# Autodesk Inventor assembly: JewlArm
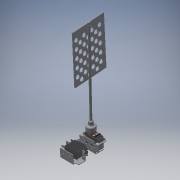
[picture p0: Inventor's stored thumbnail of the model, 180x180]
Saved by Autodesk Inventor 2017 (Build 210142000, 142)
## iProperties
Created: 2017-10-12
Part Number: JewlArm
Document SubType Name: Assembly
Designer: User
Author: User
## Documents named in this file (5)
- C:\Robotics\CAD\2017-18_CAD\Miscellaneous\JewlArm.iam
- C:\Robotics\CAD\COTSParts\Tetrix\Tetrix servo 180.ipt
- C:\Robotics\CAD\COTSParts\Tetrix\Tetrix bracket - single servo.ipt
- C:\Robotics\CAD\2017-18_CAD\FlapperSlapperPlate.ipt
- C:\Robotics\CAD\2017-18_CAD\FlapperSlapper.ipt
## Components (6 placed, 4 different names)
1. Tetrix servo 180:1 — Mate:11, Mate:12, Mate:13, Mate:21, Mate:22
2. Tetrix servo 180:2 — Mate:10, Mate:18, Mate:19, Mate:20
3. Tetrix bracket - single servo:1 — Mate:18, Mate:19, Mate:20, Flush:1, Flush:2
4. Tetrix bracket - single servo:2 — Mate:10, Mate:11, Mate:12, Mate:13, Flush:1, Flush:2
5. FlapperSlapperPlate:1 — Mate:23, Mate:24
6. FlapperSlapper:1 — Mate:21, Mate:22, Mate:23, Mate:24
## Relationships (13: Mate 11, Flush 2)
- Mate:10 (10.668 mm): Tetrix servo 180:2 ↔ Tetrix bracket - single servo:2
- Mate:11: Tetrix servo 180:1 ↔ Tetrix bracket - single servo:2
- Mate:12: Tetrix servo 180:1 ↔ Tetrix bracket - single servo:2
- Mate:13: Tetrix servo 180:1 ↔ Tetrix bracket - single servo:2
- Mate:18 (10.16 mm): Tetrix servo 180:2 ↔ Tetrix bracket - single servo:1
- Mate:19: Tetrix servo 180:2 ↔ Tetrix bracket - single servo:1
- Mate:20: Tetrix servo 180:2 ↔ Tetrix bracket - single servo:1
- Flush:1 (6.35 mm): Tetrix bracket - single servo:1 ↔ Tetrix bracket - single servo:2
- Flush:2: Tetrix bracket - single servo:1 ↔ Tetrix bracket - single servo:2
- Mate:21: Tetrix servo 180:1 ↔ FlapperSlapper:1
- Mate:22: Tetrix servo 180:1 ↔ FlapperSlapper:1
- Mate:23: FlapperSlapperPlate:1 ↔ FlapperSlapper:1
- Mate:24: FlapperSlapperPlate:1 ↔ FlapperSlapper:1
